# Autodesk Inventor assembly: Configuration 1
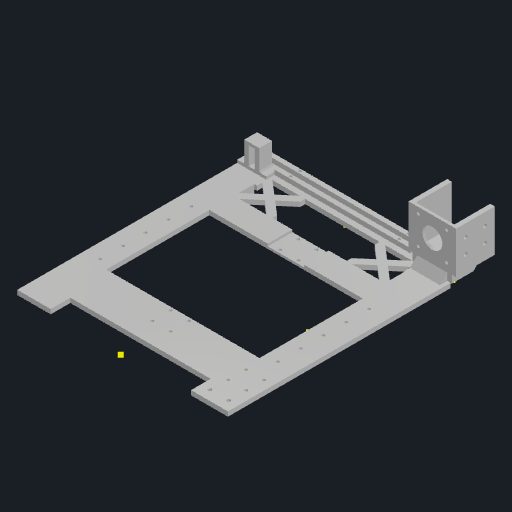
[picture p0: Inventor's stored thumbnail of the model, 512x512]
Saved by Autodesk Inventor 2026.2 (Build 302298000, 298)
## iProperties
Created: 2026-02-12
Part Number: Configuration 1
Document SubType Name: Assembly
Designer: AdminForWorker
Mass: 215.378 g
Surface Area: 1025.41 cm^2
Volume: 195.798 cm^3
Density: 1.1 g/cm^3
Title: stagex v7 new version v8
Author: AdminForWorker
## Documents named in this file (3)
- C:\Users\Alvin\OneDrive\Documents\Inventor\NCKU_Automation_Incubator_Microscope\stagex v7 new version\stagex v7 new version.iam
- C:\Users\Alvin\OneDrive\Documents\Inventor\NCKU_Automation_Incubator_Microscope\stagex v7 new version\limitswitch_bracket v2.ipt
- C:\Users\Alvin\OneDrive\Documents\Inventor\NCKU_Automation_Incubator_Microscope\stagex v7 new version\Part4.ipt
## Components (2 placed, 2 different names)
1. limitswitch_bracket v2:1 — Mate:1, Flush:2, Flush:3
2. Part4 — Mate:1, Flush:2, Flush:3
## Relationships (3: Flush 2, Mate 1)
- Mate:1: limitswitch_bracket v2:1 ↔ Part4
- Flush:2: limitswitch_bracket v2:1 ↔ Part4
- Flush:3: limitswitch_bracket v2:1 ↔ Part4
